# Autodesk Inventor assembly: Assembly1
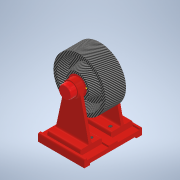
[picture p0: Inventor's stored thumbnail of the model, 180x180]
Saved by Autodesk Inventor 2021 (Build 250183000, 183)
## iProperties
Created: 2022-04-30
Part Number: Assembly1
Document SubType Name: Assembly
Designer: authe
Author: authe
## Documents named in this file (7)
- C:\Users\authe\OneDrive\Desktop\assembly\Assembly1.iam
- C:\Users\authe\OneDrive\Desktop\assembly\base.ipt
- C:\Users\authe\OneDrive\Desktop\assembly\brackett.ipt
- C:\Users\authe\OneDrive\Documents\Inventor\Content Center Files\R2021\en-US\CSN EN 28734  B\ISO 8734 - 6 x 14 - B2.ipt
- C:\Users\authe\OneDrive\Desktop\assembly\roller.ipt
- C:\Users\authe\OneDrive\Desktop\assembly\bushiing.ipt
- C:\Users\authe\OneDrive\Desktop\assembly\shaft.ipt
## Components (12 placed, 6 different names)
1. base:1 — Mate:4, Mate:5, Mate:6, Mate:7, Mate:8, Mate:9
2. brackett:2 — Mate:4, Mate:5, Insert:2, Insert:3, Mate:6, Insert:5
3. CSN EN 28734 B - replaced by CSN EN ISO 8734 6 x 14 - B:2 — Insert:3
4. CSN EN 28734 B - replaced by CSN EN ISO 8734 6 x 14 - B:3 — Insert:2
5. CSN EN 28734 B - replaced by CSN EN ISO 8734 6 x 14 - B:4 — Insert:4
6. brackett:3 — Mate:7, Mate:8, Mate:9, Insert:4, Mate:10, Mate:11, Insert:9, Insert:10
7. CSN EN 28734 B - replaced by CSN EN ISO 8734 6 x 14 - B:5 — Mate:10
8. roller:2 — Mate:11, Mate:12, Mate:14, Mate:15, Mate:16, Insert:8, Insert:11
9. bushiing:2
10. shaft:1 — Insert:5, Mate:12, Mate:14, Mate:15, Mate:16, Insert:8
11. bushiing:3 — Insert:9, Insert:10
12. bushiing:4 — Insert:11
## Relationships (20: Mate 12, Insert 8)
- Mate:4: base:1 ↔ brackett:2
- Mate:5: base:1 ↔ brackett:2
- Insert:2: brackett:2 ↔ CSN EN 28734 B - replaced by CSN EN ISO 8734 6 x 14 - B:3
- Insert:3: brackett:2 ↔ CSN EN 28734 B - replaced by CSN EN ISO 8734 6 x 14 - B:2
- Mate:6: base:1 ↔ brackett:2
- Mate:7: base:1 ↔ brackett:3
- Mate:8: base:1 ↔ brackett:3
- Mate:9: base:1 ↔ brackett:3
- Insert:4: CSN EN 28734 B - replaced by CSN EN ISO 8734 6 x 14 - B:4 ↔ brackett:3
- Mate:10: brackett:3 ↔ CSN EN 28734 B - replaced by CSN EN ISO 8734 6 x 14 - B:5
- Mate:11: brackett:3 ↔ roller:2
- Insert:5: brackett:2 ↔ shaft:1
- Mate:12: roller:2 ↔ shaft:1
- Mate:14: roller:2 ↔ shaft:1
- Mate:15: roller:2 ↔ shaft:1
- Mate:16: roller:2 ↔ shaft:1
- Insert:8: roller:2 ↔ shaft:1
- Insert:9: brackett:3 ↔ bushiing:3
- Insert:10: brackett:3 ↔ bushiing:3
- Insert:11: roller:2 ↔ bushiing:4
